# Autodesk Inventor assembly: Functioning Swerve drive (motor steering shaft)
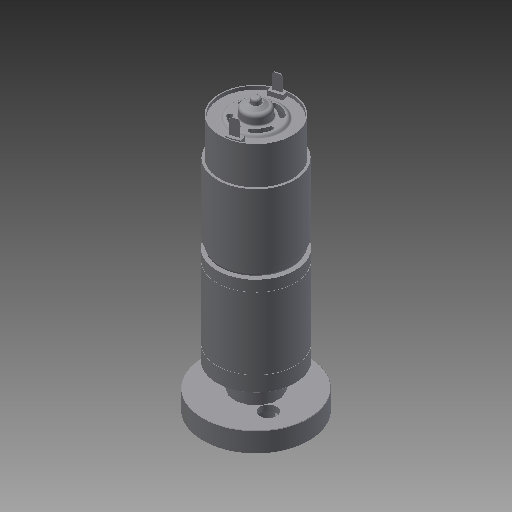
[picture p0: Inventor's stored thumbnail of the model, 512x512]
Saved by Autodesk Inventor 2019 (Build 230136000, 136)
## iProperties
Created: 2019-01-14
Part Number: Functioning Swerve drive (motor steering shaft)
Document SubType Name: Assembly
Designer: josh
Mass: 129.053 g
Surface Area: 466.568 cm^2
Volume: 129.053 cm^3
Density: 1 g/cm^3
Author: josh
## Documents named in this file (5)
- D:\Synthesis Robots\Epsilon\Functioning swerve drive sub-assemblies\Functioning Swerve drive (motor steering shaft).iam
- D:\Synthesis Robots\Epsilon\Swerve drive parts\48T 10mm bore gear.ipt
- D:\Synthesis Robots\Epsilon\Swerve drive parts\PG-71.ipt
- D:\Synthesis Robots\Epsilon\Swerve drive parts\438x406 spacer 13RS100043.ipt
- D:\Synthesis Robots\Epsilon\Swerve drive parts\375 External Self Locking Ring_98430A134.ipt
## Components (4 placed, 4 different names)
1. 48T 10mm bore gear:1
2. PG-71:1
3. 438x406 spacer 13RS100043:1
4. 375 External Self Locking Ring_98430A134:1
## Relationships (7: Mate 7)
- [Mate]: PG-71:1 ↔ 375 External Self Locking Ring_98430A134:1
- [Mate]: 48T 10mm bore gear:1 ↔ PG-71:1
- [Mate]: PG-71:1 ↔ 438x406 spacer 13RS100043:1
- [Mate]: PG-71:1 ↔ 438x406 spacer 13RS100043:1
- [Mate]: 48T 10mm bore gear:1 ↔ 438x406 spacer 13RS100043:1
- [Mate]: PG-71:1 ↔ 375 External Self Locking Ring_98430A134:1
- [Mate]: 48T 10mm bore gear:1 ↔ PG-71:1
## Named parameters: d388_d258 = 0 mm, d389_d259 = 0 mm, d340_d163 = 0 mm, d351_d266 = 0 mm, d361_d277 = 0 mm, d363_d279 = 0 mm, d364_d280 = 0 mm
